# Autodesk Inventor assembly: F624ZZ
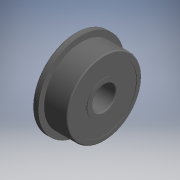
[picture p0: Inventor's stored thumbnail of the model, 180x180]
Saved by Autodesk Inventor 2017.3 (Build 213256000, 256)
## iProperties
Category: PARTsolutions
Company: NSK_RB
Part Number: F624ZZ
Catalog Web Link: www.cadenas.de
Description: Shielded Type ZZ-ZZS-
Vendor: NSK_RB
Document SubType Name: Assembly
Designer: partserver
Manufacturer: NSK_RB
Mass: 3.53 g
Surface Area: 12.5494 cm^2
Volume: 0.461029 cm^3
Density: 7.65678 g/cm^3
Title: F624ZZ
Author: Cadenas PARTsolutions
PSOL_IDENT_0: {$CADENAS_DATA\23d-libs\nsk_rb\roller_bearings\deep_groove_bb\exstra_small_miniatur_bb\metric_design
PSOL_IDENT_1: _with_flange\shielded_type_zz_zzs_1_asmtab.prj},172 {VTYP=3D},{STYP=ASSTAB},{NB=F624ZZ},{LINA=F624ZZ
PSOL_IDENT_2: },{NN=Shielded Type ZZ-ZZS},{DATE=16.07.2021 00:25:32},{GEOMDATE=04.01.2008},{VERSION=},{LINEID=230}
PSOL_IDENT_3: ,{WBVAR=},{WBNUMERIC=}  {NB=F624ZZ},{LINA=F624ZZ},{KT=DUMMY},{IDNR=},{STAN=-},{ORDER=F624ZZ},{SD=4.0
PSOL_IDENT_4: },{X=4.0},{D=13},{DD=13},{DD1=0.0},{D2=15.0},{DD2=15.0},{B=0.0},{B1=5.0},{CC1=0.0},{C2=1.0},{CC2=1.0
PSOL_IDENT_5: },{R=0.00},{R1=0.20},{DI1=6.95},{DI2=6.00},{SDE1=10.45},{SDE2=11.30},{CR1=1300},{COR1=485},{CR2=133}
PSOL_IDENT_6: ,{COR2=49.0},{LG=40000},{LO=48000},{DA=0.0},{DB=6.0},{RA=0.00},{RB=0.20},{MASS=3.53},{SC=1},{PPATH=s
PSOL_IDENT_7: hielded_type_zz_zzs_asmtpl.prj}
NB: F624ZZ
NN: Shielded Type ZZ-ZZS
NBSYN: $ORDER.
LINA: F624ZZ
CATALOG: NSK Rolling Bearing
STAN: -
ORDER: F624ZZ
SD: 4
D: 13
D2: 15
B1: 5
C2: 1
R1: 0.2
CR1: 1300
COR1: 485
CR2: 133
COR2: 49
LG: 40000
DB: 6
RB: 0.2
MASS: 3.53
SUPPLIER: NSK_RB
ARTICLENO: F624ZZ
BOMINFO: F624ZZ
CREATOR: CADENAS GmbH
## Documents named in this file (6)
- e:\temp\worker_32\temp\exporttempdir_4992_184_a5Q9n\format_0\F624ZZ.iam
- e:\temp\worker_32\temp\exporttempdir_4992_184_a5Q9n\format_0\F624ZZ Outer Ring.ipt
- e:\temp\worker_32\temp\exporttempdir_4992_184_a5Q9n\format_0\F624ZZ Inner Ring.ipt
- e:\temp\worker_32\temp\exporttempdir_4992_184_a5Q9n\format_0\F624ZZ Shield1.ipt
- e:\temp\worker_32\temp\exporttempdir_4992_184_a5Q9n\format_0\F624ZZ Ball.ipt
- e:\temp\worker_32\temp\exporttempdir_4992_184_a5Q9n\format_0\F624ZZ Shield2.ipt
## Components (11 placed, 5 different names)
1. F624ZZ Outer Ring:1 — ip_st_1_XY@1 <-> ip_st_1a_XY@2, ip_st_1_Z@1 <-> ip_st_1a_Z@2, ip_st_1_YZ@1 <-> ip_st_1a_YZ@2, ip_st_2_XY@1 <-> ip_st_1_XY@11, ip_st_2_Z@1 <-> ip_st_1_Z@11, ip_st_2_YZ@1 <-> ip_st_1_YZ@11
2. F624ZZ Inner Ring:1 — ip_st_1_XY@1 <-> ip_st_1a_XY@2, ip_st_1_Z@1 <-> ip_st_1a_Z@2, ip_st_1_YZ@1 <-> ip_st_1a_YZ@2, ip_st_2a_XY@2 <-> ip_st_1_XY@3, ip_st_2a_Z@2 <-> ip_st_1_Z@3, ip_st_2a_YZ@2 <-> ip_st_1_YZ@3, ip_st_1_1_XY@2 <-> ip_st_1_XY@4, ip_st_1_1_Z@2 <-> ip_st_1_Z@4, ip_st_1_1_YZ@2 <-> ip_st_1_YZ@4, ip_st_1_2_XY@2 <-> ip_st_1_XY@5, ip_st_1_2_Z@2 <-> ip_st_1_Z@5, ip_st_1_2_YZ@2 <-> ip_st_1_YZ@5, ip_st_1_3_XY@2 <-> ip_st_1_XY@6, ip_st_1_3_Z@2 <-> ip_st_1_Z@6, ip_st_1_3_YZ@2 <-> ip_st_1_YZ@6, ip_st_1_4_XY@2 <-> ip_st_1_XY@7, ip_st_1_4_Z@2 <-> ip_st_1_Z@7, ip_st_1_4_YZ@2 <-> ip_st_1_YZ@7, ip_st_1_5_XY@2 <-> ip_st_1_XY@8, ip_st_1_5_Z@2 <-> ip_st_1_Z@8, ip_st_1_5_YZ@2 <-> ip_st_1_YZ@8, ip_st_1_6_XY@2 <-> ip_st_1_XY@9, ip_st_1_6_Z@2 <-> ip_st_1_Z@9, ip_st_1_6_YZ@2 <-> ip_st_1_YZ@9, ip_st_1_7_XY@2 <-> ip_st_1_XY@10, ip_st_1_7_Z@2 <-> ip_st_1_Z@10, ip_st_1_7_YZ@2 <-> ip_st_1_YZ@10
3. F624ZZ Shield1:1 — ip_st_2a_XY@2 <-> ip_st_1_XY@3, ip_st_2a_Z@2 <-> ip_st_1_Z@3, ip_st_2a_YZ@2 <-> ip_st_1_YZ@3
4. F624ZZ Ball:1 — ip_st_1_1_XY@2 <-> ip_st_1_XY@4, ip_st_1_1_Z@2 <-> ip_st_1_Z@4, ip_st_1_1_YZ@2 <-> ip_st_1_YZ@4
5. F624ZZ Ball:2 — ip_st_1_2_XY@2 <-> ip_st_1_XY@5, ip_st_1_2_Z@2 <-> ip_st_1_Z@5, ip_st_1_2_YZ@2 <-> ip_st_1_YZ@5
6. F624ZZ Ball:3 — ip_st_1_3_XY@2 <-> ip_st_1_XY@6, ip_st_1_3_Z@2 <-> ip_st_1_Z@6, ip_st_1_3_YZ@2 <-> ip_st_1_YZ@6
7. F624ZZ Ball:4 — ip_st_1_4_XY@2 <-> ip_st_1_XY@7, ip_st_1_4_Z@2 <-> ip_st_1_Z@7, ip_st_1_4_YZ@2 <-> ip_st_1_YZ@7
8. F624ZZ Ball:5 — ip_st_1_5_XY@2 <-> ip_st_1_XY@8, ip_st_1_5_Z@2 <-> ip_st_1_Z@8, ip_st_1_5_YZ@2 <-> ip_st_1_YZ@8
9. F624ZZ Ball:6 — ip_st_1_6_XY@2 <-> ip_st_1_XY@9, ip_st_1_6_Z@2 <-> ip_st_1_Z@9, ip_st_1_6_YZ@2 <-> ip_st_1_YZ@9
10. F624ZZ Ball:7 — ip_st_1_7_XY@2 <-> ip_st_1_XY@10, ip_st_1_7_Z@2 <-> ip_st_1_Z@10, ip_st_1_7_YZ@2 <-> ip_st_1_YZ@10
11. F624ZZ Shield2:1 — ip_st_2_XY@1 <-> ip_st_1_XY@11, ip_st_2_Z@1 <-> ip_st_1_Z@11, ip_st_2_YZ@1 <-> ip_st_1_YZ@11
## Relationships (30: Mate 18, Angle 10, Flush 2)
- ip_st_1_XY@1 <-> ip_st_1a_XY@2 [Flush]: F624ZZ Outer Ring:1 ↔ F624ZZ Inner Ring:1
- ip_st_1_Z@1 <-> ip_st_1a_Z@2 [Mate]: F624ZZ Outer Ring:1 ↔ F624ZZ Inner Ring:1
- ip_st_1_YZ@1 <-> ip_st_1a_YZ@2 [Angle] (90 deg): F624ZZ Outer Ring:1 ↔ F624ZZ Inner Ring:1
- ip_st_2a_XY@2 <-> ip_st_1_XY@3 [Flush]: F624ZZ Inner Ring:1 ↔ F624ZZ Shield1:1
- ip_st_2a_Z@2 <-> ip_st_1_Z@3 [Mate]: F624ZZ Inner Ring:1 ↔ F624ZZ Shield1:1
- ip_st_2a_YZ@2 <-> ip_st_1_YZ@3 [Angle] (0 deg): F624ZZ Inner Ring:1 ↔ F624ZZ Shield1:1
- ip_st_1_1_XY@2 <-> ip_st_1_XY@4 [Mate]: F624ZZ Inner Ring:1 ↔ F624ZZ Ball:1
- ip_st_1_1_Z@2 <-> ip_st_1_Z@4 [Mate]: F624ZZ Inner Ring:1 ↔ F624ZZ Ball:1
- ip_st_1_1_YZ@2 <-> ip_st_1_YZ@4 [Angle] (0 deg): F624ZZ Inner Ring:1 ↔ F624ZZ Ball:1
- ip_st_1_2_XY@2 <-> ip_st_1_XY@5 [Mate]: F624ZZ Inner Ring:1 ↔ F624ZZ Ball:2
- ip_st_1_2_Z@2 <-> ip_st_1_Z@5 [Mate]: F624ZZ Inner Ring:1 ↔ F624ZZ Ball:2
- ip_st_1_2_YZ@2 <-> ip_st_1_YZ@5 [Angle] (0 deg): F624ZZ Inner Ring:1 ↔ F624ZZ Ball:2
- ip_st_1_3_XY@2 <-> ip_st_1_XY@6 [Mate]: F624ZZ Inner Ring:1 ↔ F624ZZ Ball:3
- ip_st_1_3_Z@2 <-> ip_st_1_Z@6 [Mate]: F624ZZ Inner Ring:1 ↔ F624ZZ Ball:3
- ip_st_1_3_YZ@2 <-> ip_st_1_YZ@6 [Angle] (0 deg): F624ZZ Inner Ring:1 ↔ F624ZZ Ball:3
- ip_st_1_4_XY@2 <-> ip_st_1_XY@7 [Mate]: F624ZZ Inner Ring:1 ↔ F624ZZ Ball:4
- ip_st_1_4_Z@2 <-> ip_st_1_Z@7 [Mate]: F624ZZ Inner Ring:1 ↔ F624ZZ Ball:4
- ip_st_1_4_YZ@2 <-> ip_st_1_YZ@7 [Angle] (0 deg): F624ZZ Inner Ring:1 ↔ F624ZZ Ball:4
- ip_st_1_5_XY@2 <-> ip_st_1_XY@8 [Mate]: F624ZZ Inner Ring:1 ↔ F624ZZ Ball:5
- ip_st_1_5_Z@2 <-> ip_st_1_Z@8 [Mate]: F624ZZ Inner Ring:1 ↔ F624ZZ Ball:5
- ip_st_1_5_YZ@2 <-> ip_st_1_YZ@8 [Angle] (0 deg): F624ZZ Inner Ring:1 ↔ F624ZZ Ball:5
- ip_st_1_6_XY@2 <-> ip_st_1_XY@9 [Mate]: F624ZZ Inner Ring:1 ↔ F624ZZ Ball:6
- ip_st_1_6_Z@2 <-> ip_st_1_Z@9 [Mate]: F624ZZ Inner Ring:1 ↔ F624ZZ Ball:6
- ip_st_1_6_YZ@2 <-> ip_st_1_YZ@9 [Angle] (0 deg): F624ZZ Inner Ring:1 ↔ F624ZZ Ball:6
- ip_st_1_7_XY@2 <-> ip_st_1_XY@10 [Mate]: F624ZZ Inner Ring:1 ↔ F624ZZ Ball:7
- ip_st_1_7_Z@2 <-> ip_st_1_Z@10 [Mate]: F624ZZ Inner Ring:1 ↔ F624ZZ Ball:7
- ip_st_1_7_YZ@2 <-> ip_st_1_YZ@10 [Angle] (0 deg): F624ZZ Inner Ring:1 ↔ F624ZZ Ball:7
- ip_st_2_XY@1 <-> ip_st_1_XY@11 [Mate]: F624ZZ Outer Ring:1 ↔ F624ZZ Shield2:1
- ip_st_2_Z@1 <-> ip_st_1_Z@11 [Mate]: F624ZZ Outer Ring:1 ↔ F624ZZ Shield2:1
- ip_st_2_YZ@1 <-> ip_st_1_YZ@11 [Angle] (0 deg): F624ZZ Outer Ring:1 ↔ F624ZZ Shield2:1
